# Autodesk Inventor assembly: Y-AXIS ASSEMBLY P1.2
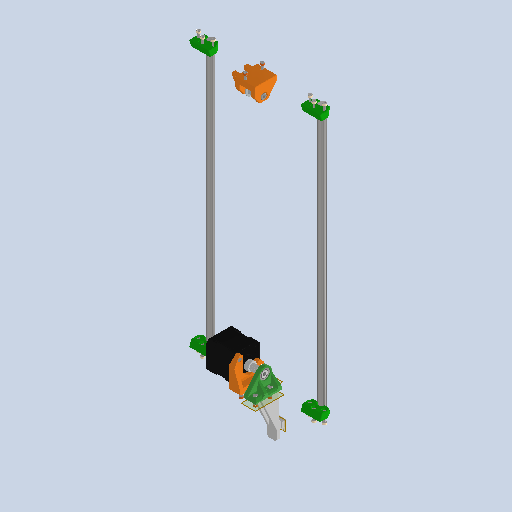
[picture p0: Inventor's stored thumbnail of the model, 512x512]
Saved by Autodesk Inventor 2023 (Build 270158000, 158)
## iProperties
Created: 2019-09-16
Part Number: Y-AXIS ASSEMBLY P1.2
Document SubType Name: Assembly
Designer: pepd9
Mass: 649.351 g
Surface Area: 943.195 cm^2
Volume: 178.893 cm^3
Density: 3.62983 g/cm^3
Author: pepd9
## Documents named in this file (19)
- D:\000 - PEPCORP CLOUD\00- Legacy\Designs\MK3PRO P1\Y-Axis\Y-AXIS ASSEMBLY P1.2.iam
- D:\000 - PEPCORP CLOUD\00- Legacy\Designs\MK3PRO P1\Y-Axis\Y-AXIS ROD.ipt
- D:\000 - PEPCORP CLOUD\00- Legacy\Designs\MK3PRO P1\Y-Axis\Y-Rod Holder.ipt
- D:\000 - PEPCORP CLOUD\00- Legacy\Designs\MK3PRO P1\COMPONENTS\M3 Nut.ipt
- D:\000 - PEPCORP CLOUD\00- Legacy\Designs\MK3PRO P1\COMPONENTS\SHCS_M3_12.ipt
- D:\000 - PEPCORP CLOUD\00- Legacy\Designs\MK3PRO P1\Y-Axis\Y-MOTOR SUPPORT.ipt
- D:\000 - PEPCORP CLOUD\00- Legacy\Designs\MK3PRO P1\Y-Axis\y-motor-holder.ipt
- D:\000 - PEPCORP CLOUD\00- Legacy\Designs\MK3PRO P1\Y-Axis\Y-AXIS STEPPER MOTOR.iam
- D:\000 - PEPCORP CLOUD\00- Legacy\Designs\MK3PRO P1\COMPONENTS\GT2_16T.ipt
- D:\000 - PEPCORP CLOUD\00- Legacy\Designs\MK3PRO P1\COMPONENTS\625 Bearing.ipt
- D:\000 - PEPCORP CLOUD\00- Legacy\Designs\MK3PRO P1\Y-Axis\y-belt-idler.ipt
- D:\000 - PEPCORP CLOUD\00- Legacy\Designs\MK3PRO P1\COMPONENTS\SHCS_M5_25.ipt
- D:\000 - PEPCORP CLOUD\00- Legacy\Designs\MK3PRO P1\COMPONENTS\M5 Nylock.ipt
- D:\000 - PEPCORP CLOUD\00- Legacy\Designs\MK3PRO P1\COMPONENTS\Idler Roller, flat.ipt
- D:\000 - PEPCORP CLOUD\00- Legacy\Designs\MK3PRO P1\COMPONENTS\SHCS_M3_8.ipt
- D:\000 - PEPCORP CLOUD\00- Legacy\Designs\MK3PRO P1\Y-Axis\YMIN-SUPPORT.ipt
- D:\000 - PEPCORP CLOUD\00- Legacy\Designs\MK3PRO P1\COMPONENTS\Small Limit Switch.iam
- D:\000 - PEPCORP CLOUD\00- Legacy\Designs\MK3PRO P1\COMPONENTS\SHCS_M2_12.ipt
- D:\000 - PEPCORP CLOUD\00- Legacy\Designs\MK3PRO P1\COMPONENTS\SHCS_M3_14.ipt
## Components (59 placed, 18 different names)
1. Y-AXIS ROD:1 — Mate:1, Mate:3, Flush:1, Mate:4, Mate:5, Mate:6, Mate:8, Flush:3
2. Y-AXIS ROD:2 — Mate:2, Mate:3, Flush:1, Mate:7, Mate:9
3. Y-Rod Holder:1 — Mate:9, Flush:4, Flush:5, Mate:11, Mate:30, Mate:31, Mate:32, Mate:39, Mate:40, Mate:41, Mate:42, Mate:43, Mate:44, Mate:146, Mate:147, Mate:148
4. Y-Rod Holder:2 — Mate:8, Mate:10, Flush:3, Flush:4, Flush:6, Mate:11, Mate:33, Mate:34, Mate:35, Mate:36, Mate:37, Mate:38, Mate:45, Mate:46, Mate:47, Flush:7, Flush:8, Mate:149, Mate:150, Mate:151
5. Y-Rod Holder:3 — Mate:6, Mate:10, Flush:2, Flush:6, Mate:18, Mate:19, Mate:20, Mate:21, Mate:22, Mate:23, Mate:24, Mate:25, Mate:26, Flush:10, Mate:155, Mate:156, Mate:157
6. Y-Rod Holder:4 — Mate:7, Flush:2, Flush:5, Mate:12, Mate:13, Mate:14, Mate:15, Mate:16, Mate:17, Mate:27, Mate:28, Mate:29, Mate:152, Mate:153, Mate:154
7. M3 Nut:1 — Mate:13, Mate:17, Mate:28
8. M3 Nut:2 — Mate:12, Mate:15, Mate:27
9. M3 Nut:3 — Mate:14, Mate:16, Mate:29
10. M3 Nut:4 — Mate:20, Mate:21, Mate:25
11. M3 Nut:5 — Mate:18, Mate:19, Mate:26
12. M3 Nut:6 — Mate:22, Mate:23, Mate:24
13. M3 Nut:7 — Mate:34, Mate:37, Mate:46
14. M3 Nut:8 — Mate:35, Mate:36, Mate:47
15. M3 Nut:9 — Mate:33, Mate:38, Mate:45
16. M3 Nut:10 — Mate:30, Mate:41, Mate:42
17. M3 Nut:11 — Mate:31, Mate:39, Mate:43
18. M3 Nut:12 — Mate:32, Mate:40, Mate:44
19. Y-MOTOR SUPPORT:1 — Flush:7, Mate:77, Mate:79, Flush:9, Mate:100, Mate:105, Mate:106, Mate:107, Mate:108, Mate:109, Mate:110, Mate:114, Mate:116, Mate:117, Mate:118, Flush:13, Mate:144
20. y-motor-holder:1 — Flush:8, Mate:79, Mate:101, Mate:102, Mate:103, Mate:104, Mate:111, Mate:112, Mate:113, Mate:115, Mate:119, Mate:120, Mate:122, Mate:124, Mate:138, Mate:140, Mate:141, Mate:142
21. GT2_16T:1 — Mate:143, Mate:144
22. 625 Bearing:1 — Mate:77, Flush:9
23. y-belt-idler:1 — Flush:10, Mate:81, Mate:82, Mate:83, Mate:86, Mate:87, Mate:90, Mate:91, Mate:92, Mate:93, Mate:94, Mate:95, Mate:96, Mate:97, Mate:98, Mate:99, Flush:11, Mate:137
24. SHCS_M5_25:1 — Mate:82, Mate:83, Mate:84, Mate:88
25. M5 Nylock:1 — Mate:84, Mate:86, Mate:87
26. Idler Roller, flat:1 — Mate:88, Mate:137
27. M3 Nut:13 — Mate:91, Mate:92, Mate:95
28. M3 Nut:14 — Mate:90, Mate:93, Mate:94
29. SHCS_M3_12:13 — Mate:96, Mate:98
30. SHCS_M3_12:14 — Mate:97, Mate:99
31. SHCS_M3_12:15 — Mate:113, Mate:119
32. SHCS_M3_12:16 — Mate:116, Mate:117
33. SHCS_M3_12:17 — Mate:115, Mate:120
34. SHCS_M3_12:18 — Mate:114, Mate:118
35. M3 Nut:15 — Mate:101, Mate:102, Mate:111
36. M3 Nut:16 — Mate:103, Mate:104, Mate:112
37. M3 Nut:17 — Mate:105, Mate:106, Mate:110
38. M3 Nut:18 — Mate:107, Mate:108, Mate:109
39. SHCS_M3_8:2 — Mate:122, Mate:124, Mate:139
40. YMIN-SUPPORT:1 — Flush:14, Mate:127, Mate:128, Mate:129, Mate:130, Mate:131, Mate:132, Mate:133
41. SHCS_M3_8:3 — Mate:127, Mate:130
42. SHCS_M3_8:4 — Mate:128, Mate:129
43. Small Limit Switch:1 [sub-assembly] — Mate:131, Mate:132, Mate:133, Mate:134, Mate:135, Mate:136, Mate:145
44. SHCS_M2_12:1 — Mate:134, Mate:145
45. SHCS_M2_12:2 — Mate:135, Mate:136
46. SHCS_M3_8:5 — Mate:141, Mate:142
47. Y-AXIS STEPPER MOTOR:1 [sub-assembly] — Mate:138, Mate:139, Mate:140, Mate:143
48. SHCS_M3_14:1 — Mate:146, Flush:15, Flush:16
49. SHCS_M3_14:2 — Mate:148, Flush:16, Flush:17
50. SHCS_M3_14:3 — Mate:147, Flush:15
51. SHCS_M3_14:4 — Mate:149, Flush:19
52. SHCS_M3_14:5 — Mate:150, Flush:18, Flush:19
53. SHCS_M3_14:6 — Mate:151, Flush:17, Flush:18
54. SHCS_M3_14:7 — Mate:152, Flush:20, Flush:21
55. SHCS_M3_14:8 — Mate:153, Flush:21
56. SHCS_M3_14:9 — Mate:154, Flush:20, Flush:22
57. SHCS_M3_14:10 — Mate:156, Flush:23, Flush:24
58. SHCS_M3_14:11 — Mate:155, Flush:22, Flush:24
59. SHCS_M3_14:12 — Mate:157, Flush:23
## Relationships (143: Mate 120, Flush 23)
- Mate:1: Y-AXIS ROD:1
- Mate:2: Y-AXIS ROD:2
- Mate:3 (170 mm): Y-AXIS ROD:1 ↔ Y-AXIS ROD:2
- Flush:1: Y-AXIS ROD:1 ↔ Y-AXIS ROD:2
- Mate:4 (-85 mm): Y-AXIS ROD:1
- Mate:5 (-203 mm): Y-AXIS ROD:1
- Mate:6: Y-AXIS ROD:1 ↔ Y-Rod Holder:3
- Mate:7: Y-AXIS ROD:2 ↔ Y-Rod Holder:4
- Mate:8: Y-AXIS ROD:1 ↔ Y-Rod Holder:2
- Mate:9: Y-AXIS ROD:2 ↔ Y-Rod Holder:1
- Mate:10 (-406.35 mm): Y-Rod Holder:2 ↔ Y-Rod Holder:3
- Flush:2: Y-Rod Holder:3 ↔ Y-Rod Holder:4
- Flush:3: Y-AXIS ROD:1 ↔ Y-Rod Holder:2
- Flush:4: Y-Rod Holder:1 ↔ Y-Rod Holder:2
- Flush:5: Y-Rod Holder:1 ↔ Y-Rod Holder:4
- Flush:6: Y-Rod Holder:2 ↔ Y-Rod Holder:3
- Mate:11 (140 mm): Y-Rod Holder:1 ↔ Y-Rod Holder:2
- Mate:12: Y-Rod Holder:4 ↔ M3 Nut:2
- Mate:13: Y-Rod Holder:4 ↔ M3 Nut:1
- Mate:14: Y-Rod Holder:4 ↔ M3 Nut:3
- Mate:15: Y-Rod Holder:4 ↔ M3 Nut:2
- Mate:16: Y-Rod Holder:4 ↔ M3 Nut:3
- Mate:17: Y-Rod Holder:4 ↔ M3 Nut:1
- Mate:18: Y-Rod Holder:3 ↔ M3 Nut:5
- Mate:19: Y-Rod Holder:3 ↔ M3 Nut:5
- Mate:20: Y-Rod Holder:3 ↔ M3 Nut:4
- Mate:21: Y-Rod Holder:3 ↔ M3 Nut:4
- Mate:22: Y-Rod Holder:3 ↔ M3 Nut:6
- Mate:23: Y-Rod Holder:3 ↔ M3 Nut:6
- Mate:24: Y-Rod Holder:3 ↔ M3 Nut:6
- Mate:25: Y-Rod Holder:3 ↔ M3 Nut:4
- Mate:26: Y-Rod Holder:3 ↔ M3 Nut:5
- Mate:27: Y-Rod Holder:4 ↔ M3 Nut:2
- Mate:28: Y-Rod Holder:4 ↔ M3 Nut:1
- Mate:29: Y-Rod Holder:4 ↔ M3 Nut:3
- Mate:30: Y-Rod Holder:1 ↔ M3 Nut:10
- Mate:31: Y-Rod Holder:1 ↔ M3 Nut:11
- Mate:32: Y-Rod Holder:1 ↔ M3 Nut:12
- Mate:33: Y-Rod Holder:2 ↔ M3 Nut:9
- Mate:34: Y-Rod Holder:2 ↔ M3 Nut:7
- Mate:35: Y-Rod Holder:2 ↔ M3 Nut:8
- Mate:36: Y-Rod Holder:2 ↔ M3 Nut:8
- Mate:37: Y-Rod Holder:2 ↔ M3 Nut:7
- Mate:38: Y-Rod Holder:2 ↔ M3 Nut:9
- Mate:39: Y-Rod Holder:1 ↔ M3 Nut:11
- Mate:40: Y-Rod Holder:1 ↔ M3 Nut:12
- Mate:41: Y-Rod Holder:1 ↔ M3 Nut:10
- Mate:42: Y-Rod Holder:1 ↔ M3 Nut:10
- Mate:43: Y-Rod Holder:1 ↔ M3 Nut:11
- Mate:44: Y-Rod Holder:1 ↔ M3 Nut:12
- Mate:45: Y-Rod Holder:2 ↔ M3 Nut:9
- Mate:46: Y-Rod Holder:2 ↔ M3 Nut:7
- Mate:47: Y-Rod Holder:2 ↔ M3 Nut:8
- Flush:7: Y-Rod Holder:2 ↔ Y-MOTOR SUPPORT:1
- Flush:8: Y-Rod Holder:2 ↔ y-motor-holder:1
- Mate:77: Y-MOTOR SUPPORT:1 ↔ 625 Bearing:1
- Mate:79 (22 mm): Y-MOTOR SUPPORT:1 ↔ y-motor-holder:1
- Flush:9: Y-MOTOR SUPPORT:1 ↔ 625 Bearing:1
- Flush:10: Y-Rod Holder:3 ↔ y-belt-idler:1
- Mate:81 (7 mm): y-belt-idler:1
- Mate:82: y-belt-idler:1 ↔ SHCS_M5_25:1
- Mate:83: y-belt-idler:1 ↔ SHCS_M5_25:1
- Mate:84: SHCS_M5_25:1 ↔ M5 Nylock:1
- Mate:86: y-belt-idler:1 ↔ M5 Nylock:1
- Mate:87: y-belt-idler:1 ↔ M5 Nylock:1
- Mate:88: SHCS_M5_25:1 ↔ Idler Roller, flat:1
- Mate:90: y-belt-idler:1 ↔ M3 Nut:14
- Mate:91: y-belt-idler:1 ↔ M3 Nut:13
- Mate:92: y-belt-idler:1 ↔ M3 Nut:13
- Mate:93: y-belt-idler:1 ↔ M3 Nut:14
- Mate:94 (0.05 mm): y-belt-idler:1 ↔ M3 Nut:14
- Mate:95 (0.05 mm): y-belt-idler:1 ↔ M3 Nut:13
- Mate:96: y-belt-idler:1 ↔ SHCS_M3_12:13
- Mate:97: y-belt-idler:1 ↔ SHCS_M3_12:14
- Mate:98 (6.35 mm): y-belt-idler:1 ↔ SHCS_M3_12:13
- Mate:99 (6.35 mm): y-belt-idler:1 ↔ SHCS_M3_12:14
- Mate:100 (-44 mm): Y-MOTOR SUPPORT:1
- Mate:101: y-motor-holder:1 ↔ M3 Nut:15
- Mate:102: y-motor-holder:1 ↔ M3 Nut:15
- Mate:103: y-motor-holder:1 ↔ M3 Nut:16
- Mate:104: y-motor-holder:1 ↔ M3 Nut:16
- Mate:105: Y-MOTOR SUPPORT:1 ↔ M3 Nut:17
- Mate:106: Y-MOTOR SUPPORT:1 ↔ M3 Nut:17
- Mate:107: Y-MOTOR SUPPORT:1 ↔ M3 Nut:18
- Mate:108: Y-MOTOR SUPPORT:1 ↔ M3 Nut:18
- Mate:109: Y-MOTOR SUPPORT:1 ↔ M3 Nut:18
- Mate:110: Y-MOTOR SUPPORT:1 ↔ M3 Nut:17
- Mate:111 (0.05 mm): y-motor-holder:1 ↔ M3 Nut:15
- Mate:112 (0.05 mm): y-motor-holder:1 ↔ M3 Nut:16
- Mate:113: y-motor-holder:1 ↔ SHCS_M3_12:15
- Mate:114: Y-MOTOR SUPPORT:1 ↔ SHCS_M3_12:18
- Mate:115: y-motor-holder:1 ↔ SHCS_M3_12:17
- Mate:116: Y-MOTOR SUPPORT:1 ↔ SHCS_M3_12:16
- Mate:117 (6.35 mm): Y-MOTOR SUPPORT:1 ↔ SHCS_M3_12:16
- Mate:118 (6.35 mm): Y-MOTOR SUPPORT:1 ↔ SHCS_M3_12:18
- Mate:119 (6.35 mm): y-motor-holder:1 ↔ SHCS_M3_12:15
- Mate:120 (6.35 mm): y-motor-holder:1 ↔ SHCS_M3_12:17
- Mate:122: y-motor-holder:1 ↔ SHCS_M3_8:2
- Mate:124: y-motor-holder:1 ↔ SHCS_M3_8:2
- Flush:11 (-2.96 mm): y-belt-idler:1
- Flush:13 (6.35 mm): Y-MOTOR SUPPORT:1
- Flush:14: YMIN-SUPPORT:1
- Mate:127: YMIN-SUPPORT:1 ↔ SHCS_M3_8:3
- Mate:128: YMIN-SUPPORT:1 ↔ SHCS_M3_8:4
- Mate:129: YMIN-SUPPORT:1 ↔ SHCS_M3_8:4
- Mate:130: YMIN-SUPPORT:1 ↔ SHCS_M3_8:3
- Mate:131: YMIN-SUPPORT:1 ↔ Small Limit Switch:1
- Mate:132: YMIN-SUPPORT:1 ↔ Small Limit Switch:1
- Mate:133: YMIN-SUPPORT:1 ↔ Small Limit Switch:1
- Mate:134: Small Limit Switch:1 ↔ SHCS_M2_12:1
- Mate:135: Small Limit Switch:1 ↔ SHCS_M2_12:2
- Mate:136: Small Limit Switch:1 ↔ SHCS_M2_12:2
- Mate:137 (0.5 mm): y-belt-idler:1 ↔ Idler Roller, flat:1
- Mate:138: y-motor-holder:1 ↔ Y-AXIS STEPPER MOTOR:1
- Mate:139: SHCS_M3_8:2 ↔ Y-AXIS STEPPER MOTOR:1
- Mate:140: y-motor-holder:1 ↔ Y-AXIS STEPPER MOTOR:1
- Mate:141: y-motor-holder:1 ↔ SHCS_M3_8:5
- Mate:142: y-motor-holder:1 ↔ SHCS_M3_8:5
- Mate:143: GT2_16T:1 ↔ Y-AXIS STEPPER MOTOR:1
- Mate:144 (1 mm): Y-MOTOR SUPPORT:1 ↔ GT2_16T:1
- Mate:145: Small Limit Switch:1 ↔ SHCS_M2_12:1
- Mate:146: Y-Rod Holder:1 ↔ SHCS_M3_14:1
- Mate:147: Y-Rod Holder:1 ↔ SHCS_M3_14:3
- Mate:148: Y-Rod Holder:1 ↔ SHCS_M3_14:2
- Flush:15: SHCS_M3_14:1 ↔ SHCS_M3_14:3
- Flush:16: SHCS_M3_14:1 ↔ SHCS_M3_14:2
- Mate:149: Y-Rod Holder:2 ↔ SHCS_M3_14:4
- Mate:150: Y-Rod Holder:2 ↔ SHCS_M3_14:5
- Mate:151: Y-Rod Holder:2 ↔ SHCS_M3_14:6
- Flush:17: SHCS_M3_14:2 ↔ SHCS_M3_14:6
- Flush:18: SHCS_M3_14:5 ↔ SHCS_M3_14:6
- Flush:19: SHCS_M3_14:4 ↔ SHCS_M3_14:5
- Mate:152: Y-Rod Holder:4 ↔ SHCS_M3_14:7
- Mate:153: Y-Rod Holder:4 ↔ SHCS_M3_14:8
- Mate:154: Y-Rod Holder:4 ↔ SHCS_M3_14:9
- Flush:20: SHCS_M3_14:7 ↔ SHCS_M3_14:9
- Flush:21: SHCS_M3_14:7 ↔ SHCS_M3_14:8
- Mate:155: Y-Rod Holder:3 ↔ SHCS_M3_14:11
- Mate:156: Y-Rod Holder:3 ↔ SHCS_M3_14:10
- Mate:157: Y-Rod Holder:3 ↔ SHCS_M3_14:12
- Flush:22: SHCS_M3_14:9 ↔ SHCS_M3_14:11
- Flush:23: SHCS_M3_14:10 ↔ SHCS_M3_14:12
- Flush:24: SHCS_M3_14:10 ↔ SHCS_M3_14:11
